# Autodesk Inventor assembly: Box
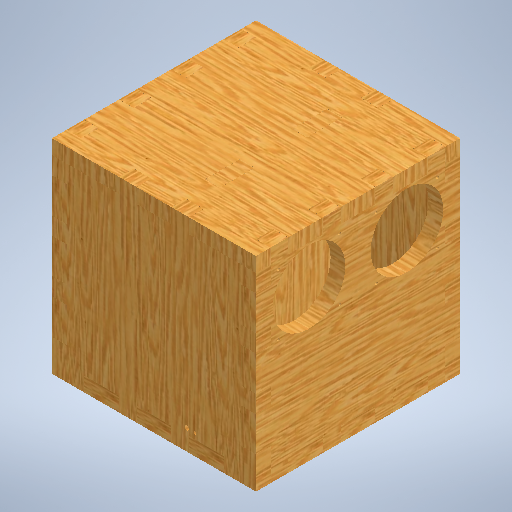
[picture p0: Inventor's stored thumbnail of the model, 512x512]
Saved by Autodesk Inventor 2025.3 (Build 293356000, 356)
## iProperties
Created: 2025-12-22
Part Number: Box
Document SubType Name: Assembly
Designer: Balint
Author: Balint
## Documents named in this file (8)
- C:\Users\Balint\3D\2.1LoudBox\Box.iam
- C:\Users\Balint\3D\2.1LoudBox\BBox.ipt
- C:\Users\Balint\3D\2.1LoudBox\FBox.ipt
- C:\Users\Balint\3D\2.1LoudBox\BABox.ipt
- C:\Users\Balint\3D\2.1LoudBox\SBox.ipt
- C:\Users\Balint\3D\2.1LoudBox\S2Box.ipt
- C:\Users\Balint\3D\2.1LoudBox\TBox.ipt
- C:\Users\Balint\3D\2.1LoudBox\IBox.ipt
## Components (7 placed, 7 different names)
1. BBox:1 — Mate:1, Mate:2, Mate:3, Mate:4, Mate:5, Mate:7, Mate:8, Flush:3
2. FBox:1 — Mate:1, Mate:2, Mate:6, Mate:9, Mate:10, Mate:11
3. BABox:1 — Mate:3, Mate:4, Mate:5, Flush:1, Flush:2
4. SBox:1 — Flush:1, Mate:6, Mate:7, Mate:8, Mate:12
5. S2Box:1 — Mate:9, Mate:10
6. TBox:1 — Flush:2, Mate:11, Mate:12
7. IBox:1 — Flush:3
## Relationships (15: Mate 12, Flush 3)
- Mate:1: BBox:1 ↔ FBox:1
- Mate:2: BBox:1 ↔ FBox:1
- Mate:3: BBox:1 ↔ BABox:1
- Mate:4: BBox:1 ↔ BABox:1
- Mate:5: BBox:1 ↔ BABox:1
- Flush:1: BABox:1 ↔ SBox:1
- Mate:6: FBox:1 ↔ SBox:1
- Mate:7: BBox:1 ↔ SBox:1
- Mate:8: BBox:1 ↔ SBox:1
- Mate:9: FBox:1 ↔ S2Box:1
- Mate:10: FBox:1 ↔ S2Box:1
- Flush:2: BABox:1 ↔ TBox:1
- Mate:11: FBox:1 ↔ TBox:1
- Mate:12: SBox:1 ↔ TBox:1
- Flush:3: BBox:1 ↔ IBox:1
